# Autodesk Inventor assembly: Mark 6 - Output Shaft
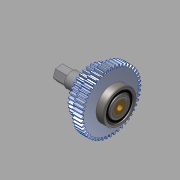
[picture p0: Inventor's stored thumbnail of the model, 180x180]
Saved by Autodesk Inventor 2013 (Build 170138000, 138)
## iProperties
Created: 2013-10-31
Part Number: Mark 6 - Output Shaft
Document SubType Name: Assembly
Designer: grtstudent
Author: grtstudent
## Documents named in this file (8)
- C:\Users\grtstudent\Desktop\Mark 6 Final Preseason\Mark 6 - Output Shaft.iam
- C:\Users\grtstudent\Desktop\Mark 6 Final Preseason\Bearings\R10-2RS.ipt
- C:\Users\grtstudent\Desktop\Mark 6 Final Preseason\Shafts\Output Shaft\35T 20DP - .188 Ball Shifting Bore.ipt
- C:\Users\grtstudent\Desktop\Mark 6 Final Preseason\Shafts\Output Shaft\48T 20DP - .188 Ball Shifting Bore.ipt
- C:\Users\grtstudent\Desktop\Mark 6 Final Preseason\Shafts\Output Shaft\Output Shaft Bushing.ipt
- C:\Users\grtstudent\Desktop\Mark 6 Final Preseason\Shafts\Output Shaft\Output Shaft.ipt
- C:\Users\grtstudent\Desktop\Mark 6 Final Preseason\Bearings\R10-Open.ipt
- C:\Users\grtstudent\Desktop\Mark 6 Final Preseason\Bearings\Thrust Bearing Washer - .6250 Bore.ipt
## Components (10 placed, 7 different names)
1. R10-2RS:1 — Mate:1, Mate:2
2. R10-2RS:2 — Mate:18, Mate:19
3. 35T 20DP - .188 Ball Shifting Bore:1 — Mate:6, Mate:7, Mate:15
4. 48T 20DP - .188 Ball Shifting Bore:1 — Mate:8, Mate:9, Mate:17
5. Output Shaft Bushing:1 — Mate:3, Mate:4
6. Output Shaft:1 — Mate:1, Mate:2, Mate:3, Mate:4, Mate:10, Mate:11, Mate:12, Mate:13, Mate:14, Mate:18
7. R10-Open:1 — Mate:6, Mate:7, Mate:11, Mate:12
8. R10-Open:2 — Mate:8, Mate:9, Mate:10, Mate:16
9. Thrust Bearing Washer - .6250 Bore:1 — Mate:13, Mate:17, Mate:19
10. Thrust Bearing Washer - .6250 Bore:2 — Mate:14, Mate:15, Mate:16
## Relationships (18: Mate 18)
- Mate:1: R10-2RS:1 ↔ Output Shaft:1
- Mate:2: R10-2RS:1 ↔ Output Shaft:1
- Mate:3: Output Shaft Bushing:1 ↔ Output Shaft:1
- Mate:4: Output Shaft Bushing:1 ↔ Output Shaft:1
- Mate:6: 35T 20DP - .188 Ball Shifting Bore:1 ↔ R10-Open:1
- Mate:7: 35T 20DP - .188 Ball Shifting Bore:1 ↔ R10-Open:1
- Mate:8: 48T 20DP - .188 Ball Shifting Bore:1 ↔ R10-Open:2
- Mate:9: 48T 20DP - .188 Ball Shifting Bore:1 ↔ R10-Open:2
- Mate:10: Output Shaft:1 ↔ R10-Open:2
- Mate:11: Output Shaft:1 ↔ R10-Open:1
- Mate:12: Output Shaft:1 ↔ R10-Open:1
- Mate:13: Output Shaft:1 ↔ Thrust Bearing Washer - .6250 Bore:1
- Mate:14: Output Shaft:1 ↔ Thrust Bearing Washer - .6250 Bore:2
- Mate:15: 35T 20DP - .188 Ball Shifting Bore:1 ↔ Thrust Bearing Washer - .6250 Bore:2
- Mate:16: R10-Open:2 ↔ Thrust Bearing Washer - .6250 Bore:2
- Mate:17: 48T 20DP - .188 Ball Shifting Bore:1 ↔ Thrust Bearing Washer - .6250 Bore:1
- Mate:18: R10-2RS:2 ↔ Output Shaft:1
- Mate:19: R10-2RS:2 ↔ Thrust Bearing Washer - .6250 Bore:1
